# Autodesk Inventor assembly: złożenie
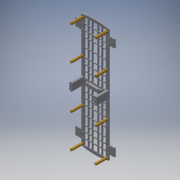
[picture p0: Inventor's stored thumbnail of the model, 180x180]
Saved by Autodesk Inventor 2016 (Build 200138000, 138)
## iProperties
Created: 2016-09-21
Part Number: złożenie
Document SubType Name: Assembly
Designer: Jakub
Author: Jakub
## Documents named in this file (4)
- C:\Users\Jakub\Documents\DATA BANK\Projekty\Dron\Enix\złożenie.iam
- C:\Users\Jakub\Documents\DATA BANK\Projekty\Dron\Enix\front\f1.ipt
- C:\Users\Jakub\Documents\DATA BANK\Projekty\Dron\Enix\common\30mm_dist.ipt
- C:\Users\Jakub\Documents\DATA BANK\Projekty\Dron\Enix\body\b1.ipt
## Components (12 placed, 3 different names)
1. f1:1 — Mate:1, Mate:2, Mate:3, Mate:4, Mate:5, Mate:8, Mate:9, Mate:13, Mate:15
2. f1:2 — Mate:1, Mate:2, Mate:3, Mate:6, Mate:7, Mate:10, Mate:11, Mate:12, Mate:14
3. 30mm_dist:1 — Mate:11
4. 30mm_dist:2 — Mate:10
5. 30mm_dist:3 — Mate:9
6. 30mm_dist:4 — Mate:8
7. 30mm_dist:5 — Mate:4
8. 30mm_dist:6 — Mate:5
9. 30mm_dist:7 — Mate:6
10. 30mm_dist:8 — Mate:7
11. b1:1 — Mate:14, Mate:15
12. b1:2 — Mate:12, Mate:13
## Relationships (15: Mate 15)
- Mate:1: f1:1 ↔ f1:2
- Mate:2: f1:1 ↔ f1:2
- Mate:3: f1:1 ↔ f1:2
- Mate:4: f1:1 ↔ 30mm_dist:5
- Mate:5: f1:1 ↔ 30mm_dist:6
- Mate:6: f1:2 ↔ 30mm_dist:7
- Mate:7: f1:2 ↔ 30mm_dist:8
- Mate:8: f1:1 ↔ 30mm_dist:4
- Mate:9: f1:1 ↔ 30mm_dist:3
- Mate:10: f1:2 ↔ 30mm_dist:2
- Mate:11: f1:2 ↔ 30mm_dist:1
- Mate:12: f1:2 ↔ b1:2
- Mate:13: f1:1 ↔ b1:2
- Mate:14: f1:2 ↔ b1:1
- Mate:15: f1:1 ↔ b1:1
